# Autodesk Inventor assembly: Rotation Lab Assembly
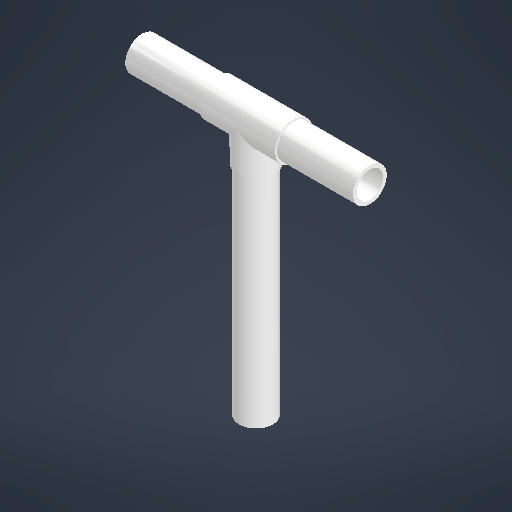
[picture p0: Inventor's stored thumbnail of the model, 512x512]
Saved by Autodesk Inventor 2027 (Build 310192000, 192)
## iProperties
Created: 2026-04-30
Part Number: Rotation Lab Assembly
Document SubType Name: Assembly
Designer: bhoga
Mass: 70.3313 g
Surface Area: 472.43 cm^2
Volume: 50.2367 cm^3
Density: 1.4 g/cm^3
Author: bhoga
## Documents named in this file (4)
- C:\Users\bhoga\OneDrive\Documents\Inventor\Content Center Files\R2027\Rotation Lab Assembly.iam
- C:\Users\bhoga\OneDrive\Documents\Inventor\Content Center Files\R2027\Connector.ipt
- C:\Users\bhoga\OneDrive\Documents\Inventor\Content Center Files\R2027\Horizontal Pipe.ipt
- C:\Users\bhoga\OneDrive\Documents\Inventor\Content Center Files\R2027\Vertical Pipe.ipt
## Components (3 placed, 3 different names)
1. Connector:1 — Rigid:1, Rigid:2
2. Horizontal Pipe:1 — Rigid:2
3. Vertical Pipe:1 — Rigid:1
## Relationships (2: WeldJoint 2)
- Rigid:1 [WeldJoint] (6.35 mm): Connector:1 ↔ Vertical Pipe:1
- Rigid:2 [WeldJoint]: Connector:1 ↔ Horizontal Pipe:1
